# Autodesk Inventor assembly: Delivery
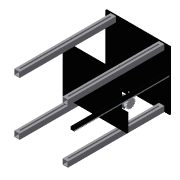
[picture p0: Inventor's stored thumbnail of the model, 180x180]
Saved by Autodesk Inventor 2016 (Build 200138000, 138)
## iProperties
Created: 2016-04-03
Part Number: Delivery
Document SubType Name: Assembly
Designer: Ariana
Author: Ariana
## Documents named in this file (9)
- C:\Users\Ariana\Downloads\Capstone CAD\Capstone CAD\Delivery\Delivery.iam
- C:\Users\Ariana\Downloads\Capstone CAD\Capstone CAD\Delivery\Base.ipt
- C:\Users\Ariana\Downloads\Capstone CAD\Capstone CAD\Delivery\Rail.ipt
- C:\Users\Ariana\Downloads\Capstone CAD\Capstone CAD\Delivery\Board.ipt
- C:\Users\Ariana\Downloads\Capstone CAD\Capstone CAD\Delivery\Bolt.ipt
- C:\Users\Ariana\Downloads\Capstone CAD\Capstone CAD\Delivery\Drive.iam
- C:\Users\Ariana\Downloads\Capstone CAD\Capstone CAD\Pinion Gear.ipt
- C:\Users\Ariana\Downloads\Capstone CAD\Capstone CAD\Motor.ipt
- C:\Users\Ariana\Downloads\Capstone CAD\Capstone CAD\Delivery\Motor mount.ipt
## Components (14 placed, 8 different names)
1. Base:1 — Mate:1, Mate:2, Flush:1, Flush:2, Flush:3, Mate:3, Flush:4, Mate:4, Flush:5, Flush:7, Mate:5, Mate:6, Mate:16
2. Rail:1 — Flush:2, Flush:3, Mate:3, Flush:6, Flush:10, Flush:14
3. Rail:2 — Flush:6, Flush:7, Mate:5, Flush:9, Mate:9
4. Rail:3 — Flush:4, Mate:4, Flush:5, Flush:8, Mate:7, Mate:13
5. Rail:4 — Mate:6, Flush:8, Flush:9
6. Board:1 — Mate:7, Flush:10, Mate:8, Tangent:1, Mate:11, Mate:12, Tangent:2, Mate:15, Flush:18, Tangent:4, Angle:1
7. Bolt:1 — Mate:10, Mate:11
8. Bolt:2 — Mate:12, Mate:13, Tangent:2, Mate:14
9. Bolt:3 — Mate:8, Mate:9, Tangent:1, Mate:10
10. Bolt:4 — Mate:14, Mate:15
11. Drive:1 [sub-assembly] — Mate:16, Flush:18, Flush:12, Tangent:3, Flush:14
12. Pinion Gear:1 — Mate:18, Mate:20, Flush:12, Tangent:3
13. Motor:1 — Mate:18, Mate:20, Tangent:4, Mate:21, Flush:13
14. Motor mount:1 — Mate:21, Flush:13, Angle:1
## Relationships (38: Mate 19, Flush 14, Tangent 4, Angle 1)
- Mate:1: Base:1
- Mate:2: Base:1
- Flush:1: Base:1
- Flush:2: Base:1 ↔ Rail:1
- Flush:3 (25.4 mm): Base:1 ↔ Rail:1
- Mate:3: Base:1 ↔ Rail:1
- Flush:4: Base:1 ↔ Rail:3
- Mate:4: Base:1 ↔ Rail:3
- Flush:5 (25.4 mm): Base:1 ↔ Rail:3
- Flush:6: Rail:1 ↔ Rail:2
- Flush:7: Base:1 ↔ Rail:2
- Mate:5: Base:1 ↔ Rail:2
- Mate:6: Base:1 ↔ Rail:4
- Flush:8: Rail:3 ↔ Rail:4
- Flush:9: Rail:2 ↔ Rail:4
- Mate:7: Rail:3 ↔ Board:1
- Flush:10 (-25.4 mm): Rail:1 ↔ Board:1
- Mate:8: Board:1 ↔ Bolt:3
- Mate:9 (3.175 mm): Rail:2 ↔ Bolt:3
- Tangent:1: Board:1 ↔ Bolt:3
- Mate:10: Bolt:1 ↔ Bolt:3
- Mate:11: Board:1 ↔ Bolt:1
- Mate:12: Board:1 ↔ Bolt:2
- Mate:13 (3.175 mm): Rail:3 ↔ Bolt:2
- Tangent:2: Board:1 ↔ Bolt:2
- Mate:14: Bolt:2 ↔ Bolt:4
- Mate:15: Board:1 ↔ Bolt:4
- Mate:16: Base:1 ↔ Drive:1
- Flush:18: Board:1 ↔ Drive:1
- Mate:18: Pinion Gear:1 ↔ Motor:1
- Mate:20: Pinion Gear:1 ↔ Motor:1
- Flush:12: Drive:1 ↔ Pinion Gear:1
- Tangent:3: Drive:1 ↔ Pinion Gear:1
- Tangent:4: Board:1 ↔ Motor:1
- Mate:21: Motor:1 ↔ Motor mount:1
- Flush:13 (25.4 mm): Motor:1 ↔ Motor mount:1
- Angle:1 (0 deg): Board:1 ↔ Motor mount:1
- Flush:14 (102.846 mm): Rail:1 ↔ Drive:1
